# Autodesk Inventor assembly: CimpleLeft
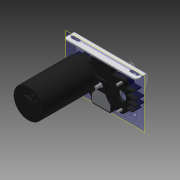
[picture p0: Inventor's stored thumbnail of the model, 180x180]
Saved by Autodesk Inventor 2015 SP1 (Build 190203100, 203)
## iProperties
Created: 2015-01-23
Part Number: CimpleLeft
Document SubType Name: Assembly
Designer: pltwe4
Author: Unknown
Title: S:/Products/Gearboxes Spur Single Stage/Single Stage Toughbox/CIMple Box.stp
Organization: Unknown
Description: Unknown
Sending System: Unknown
Preprocessor: XStep 1.0
Author: pltwe4
## Documents named in this file (16)
- E:\CAD Models\Robotics BenT\CimpleLeft.iam
- E:\CAD Models\Robotics BenT\Imported Components\CIMple Box\Single_d01.ipt
- E:\CAD Models\Robotics BenT\Imported Components\CIMple Box\10-32x0625_shcs.ipt
- E:\CAD Models\Robotics BenT\Imported Components\CIMple Box\r6zz.ipt
- E:\CAD Models\Robotics BenT\Imported Components\CIMple Box\Single_d03.ipt
- E:\CAD Models\Robotics BenT\Imported Components\CIMple Box\Single_d04.ipt
- E:\CAD Models\Robotics BenT\Imported Components\CIMple Box\Single_d02.ipt
- E:\CAD Models\Robotics BenT\Imported Components\CIMple Box\fr-8-zz.ipt
- E:\CAD Models\Robotics BenT\Imported Components\CIMple Box\CIM motor.ipt
- E:\CAD Models\Robotics BenT\Imported Components\CIMple Box\8mm_spring_clip.ipt
- E:\CAD Models\Robotics BenT\Imported Components\CIMple Box\250_washer.ipt
- E:\CAD Models\Robotics BenT\Imported Components\CIMple Box\14-20x0500_bhcs.ipt
- E:\CAD Models\Robotics BenT\Imported Components\CIMple Box\Single_d05.ipt
- E:\CAD Models\Robotics BenT\Imported Components\CIMple Box\CIMple Box Sticker.ipt
- E:\CAD Models\Robotics BenT\Imported Components\CIMple Box\10-32_nylock_nut.ipt
- E:\CAD Models\Robotics BenT\Imported Components\CIMple Box\125x124x700_key.ipt
## Components (23 placed, 15 different names)
1. Single_d01 — Mate:1, Mate:2, Mate:3
2. 10-32x0625_shcs:1
3. 10-32x0625_shcs:2
4. 10-32x0625_shcs:3
5. 10-32x0625_shcs:4
6. 10-32x0625_shcs:5
7. 10-32x0625_shcs:7
8. r6zz
9. Single_d03
10. Single_d04
11. Single_d02
12. fr-8-zz
13. CIM motor — Mate:1, Mate:2, Mate:3, Mate:4, Mate:5, Mate:7
14. 8mm_spring_clip:1 — Mate:6, Mate:7
15. 250_washer
16. 14-20x0500_bhcs
17. Single_d05:1 — Mate:4, Mate:5, Mate:6
18. CIMple Box Sticker
19. 10-32_nylock_nut
20. 10-32_nylock_nut:1
21. 10-32_nylock_nut:2
22. 10-32_nylock_nut:3
23. 125x124x700_key
## Relationships (7: Mate 7)
- Mate:1: Single_d01 ↔ CIM motor
- Mate:2: Single_d01 ↔ CIM motor
- Mate:3: Single_d01 ↔ CIM motor
- Mate:4: CIM motor ↔ Single_d05:1
- Mate:5: CIM motor ↔ Single_d05:1
- Mate:6: 8mm_spring_clip:1 ↔ Single_d05:1
- Mate:7: CIM motor ↔ 8mm_spring_clip:1
